# Autodesk Inventor assembly: camWithRubberBand
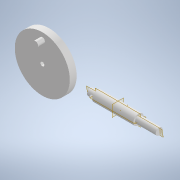
[picture p0: Inventor's stored thumbnail of the model, 180x180]
Saved by Autodesk Inventor 2020.2 (Build 242310000, 310)
## iProperties
Created: 2020-01-12
Part Number: camWithRubberBand
Document SubType Name: Assembly
Designer: robst
Author: robst
## Documents named in this file (5)
- C:\git\CAD-Development\robSteele\2020BallTriggerMechanism\camWithRubberBand.iam
- C:\git\CAD-Development\robSteele\2020LongRobotBase\camWheel.ipt
- C:\git\CAD-Development\robSteele\2020LongRobotBase\cylinderForKicker.ipt
- C:\git\CAD-Development\robSteele\2020BallTriggerMechanism\plungerForTrigger.ipt
- C:\git\CAD-Development\robSteele\2020BallTriggerMechanism\camPost.ipt
## Components (4 placed, 4 different names)
1. camWheel:1 — Flush:2, Mate:1, Flush:3, Insert:2
2. cylinderForKicker:1 — Flush:2, Mate:1, Insert:1, Flush:3
3. plungerForTrigger:1 — Insert:1
4. camPost:1 — Insert:2
## Relationships (5: Flush 2, Insert 2, Mate 1)
- Flush:2: camWheel:1 ↔ cylinderForKicker:1
- Mate:1 (203.2 mm): camWheel:1 ↔ cylinderForKicker:1
- Insert:1 (76.2 mm): cylinderForKicker:1 ↔ plungerForTrigger:1
- Flush:3: camWheel:1 ↔ cylinderForKicker:1
- Insert:2: camWheel:1 ↔ camPost:1
